# Autodesk Inventor assembly: hubRingJig
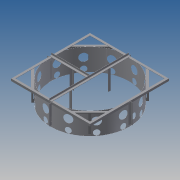
[picture p0: Inventor's stored thumbnail of the model, 180x180]
Saved by Autodesk Inventor 2014 SP1 (Build 180222100, 222)
## iProperties
Created: 2014-12-02
Part Number: hubRingJig
Document SubType Name: Assembly
Designer: Dave
Author: Dave
## Documents named in this file (10)
- C:\Users\Dave\Desktop\hera-cad\jigs\hubRingJig.iam
- C:\Users\Dave\Desktop\hera-cad\jigs\hubRingJigOuter.ipt
- C:\Users\Dave\Desktop\hera-cad\jigs\hubRingJigCross.ipt
- C:\Users\Dave\Desktop\hera-cad\jigs\hubRingJigEdgeVert.ipt
- C:\Users\Dave\Desktop\hera-cad\jigs\hubRingJigCrossShort.ipt
- C:\Users\Dave\Desktop\hera-cad\jigs\hubRingJig45.ipt
- C:\Users\Dave\Desktop\hera-cad\jigs\hubRingJigInnerVert.ipt
- C:\Users\Dave\Desktop\hera-cad\hub\ringOuter.ipt
- C:\Users\Dave\Desktop\hera-cad\hub\ringInner.ipt
- C:\Users\Dave\Desktop\hera-cad\jigs\hubRingInnerWoodFull.ipt
## Components (25 placed, 9 different names)
1. hubRingJigCross:1 — Mate:1, Flush:1, Flush:2, Flush:3, Mate:3, Flush:5, Flush:6, Flush:8, Insert:1, Insert:2, Insert:3
2. hubRingJigCrossShort:1 — Mate:3, Flush:5, Flush:6, Mate:7, Flush:7
3. ringOuter:1 — Insert:1
4. ringInner:1 — Insert:2
5. hubRingInnerWoodFull:1 — Mate:8, Mate:9, Mate:10
6. hubRingInnerWoodFull:2 — Mate:8, Mate:9, Mate:10, Insert:3
7. hubRingJigOuter:1 — Mate:1, Flush:1, Flush:2, Mate:4, Mate:6
8. hubRingJigOuter:2 — Mate:2, Flush:4, Mate:5
9. hubRingJigOuter:3
10. hubRingJigOuter:4
11. hubRingJigEdgeVert:1 — Mate:2, Flush:3, Flush:4
12. hubRingJigEdgeVert:2
13. hubRingJigEdgeVert:3
14. hubRingJigEdgeVert:4
15. hubRingJigEdgeVert:5
16. hubRingJigEdgeVert:6
17. hubRingJigEdgeVert:7
18. hubRingJigEdgeVert:8
19. hubRingJig45:1 — Mate:4, Mate:5, Mate:6
20. hubRingJig45:2
21. hubRingJig45:3
22. hubRingJig45:4
23. hubRingJigInnerVert:1 — Mate:7, Flush:7, Flush:8
24. hubRingJigInnerVert:2
25. hubRingJigInnerVert:4
## Component patterns: (4 elements, first: hubRingJigOuter:1), (8 elements, first: hubRingJigEdgeVert:1), (4 elements, first: hubRingJig45:1), (4 elements, first: hubRingJigInnerVert:1)
## Relationships (21: Mate 10, Flush 8, Insert 3)
- Mate:1: hubRingJigCross:1 ↔ hubRingJigOuter:1
- Flush:1 (-447.04 mm): hubRingJigCross:1 ↔ hubRingJigOuter:1
- Flush:2: hubRingJigCross:1 ↔ hubRingJigOuter:1
- Mate:2: hubRingJigOuter:2 ↔ hubRingJigEdgeVert:1
- Flush:3: hubRingJigCross:1 ↔ hubRingJigEdgeVert:1
- Flush:4 (-5.715 mm): hubRingJigOuter:2 ↔ hubRingJigEdgeVert:1
- Mate:3: hubRingJigCross:1 ↔ hubRingJigCrossShort:1
- Flush:5: hubRingJigCross:1 ↔ hubRingJigCrossShort:1
- Flush:6 (-447.04 mm): hubRingJigCross:1 ↔ hubRingJigCrossShort:1
- Mate:4: hubRingJigOuter:1 ↔ hubRingJig45:1
- Mate:5: hubRingJigOuter:2 ↔ hubRingJig45:1
- Mate:6: hubRingJigOuter:1 ↔ hubRingJig45:1
- Mate:7: hubRingJigCrossShort:1 ↔ hubRingJigInnerVert:1
- Flush:7: hubRingJigCrossShort:1 ↔ hubRingJigInnerVert:1
- Flush:8 (213.36 mm): hubRingJigCross:1 ↔ hubRingJigInnerVert:1
- Insert:1 (-259.08 mm): hubRingJigCross:1 ↔ ringOuter:1
- Insert:2 (-259.08 mm): hubRingJigCross:1 ↔ ringInner:1
- Mate:8: hubRingInnerWoodFull:1 ↔ hubRingInnerWoodFull:2
- Mate:9: hubRingInnerWoodFull:1 ↔ hubRingInnerWoodFull:2
- Mate:10: hubRingInnerWoodFull:1 ↔ hubRingInnerWoodFull:2
- Insert:3 (-254 mm): hubRingJigCross:1 ↔ hubRingInnerWoodFull:2
## Named parameters: hubAngleThickness = 2.54 mm, hubAngleWidth1 = 25.4 mm, hubAngleWidth2 = 25.4 mm, hubOuterDiam = 914.4 mm, hubInnerDiam = 457.2 mm, hubRingThickness = 1.524 mm, hubCentralHoleOffset = 12.7 mm
